# Autodesk Inventor assembly: kamerica
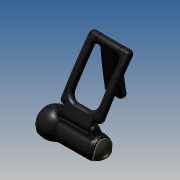
[picture p0: Inventor's stored thumbnail of the model, 180x180]
Saved by Autodesk Inventor 2012 (Build 160160000, 160)
## iProperties
Created: 2011-11-30
Part Number: kamerica
Document SubType Name: Assembly
Designer: slazh bliskovic
Author: slazh bliskovic
## Documents named in this file (12)
- C:\Users\BOZIDAR\Documents\Inventor\quickcam pro 9000\kamerica.iam
- C:\Users\BOZIDAR\Documents\Inventor\quickcam pro 9000\kamerica.ipt
- C:\Users\BOZIDAR\Documents\Inventor\quickcam pro 9000\gornji shiny dio.ipt
- C:\Users\BOZIDAR\Documents\Inventor\quickcam pro 9000\objektiv.ipt
- C:\Users\BOZIDAR\Documents\Inventor\quickcam pro 9000\unutrasnja plastika.ipt
- C:\Users\BOZIDAR\Documents\Inventor\quickcam pro 9000\staklence.ipt
- C:\Users\BOZIDAR\Documents\Inventor\quickcam pro 9000\svjetlasce.ipt
- C:\Users\BOZIDAR\Documents\Inventor\quickcam pro 9000\staklo.ipt
- C:\Users\BOZIDAR\Documents\Inventor\Content Center Files\R2012\en-US\IFI 513(1)\IFI 513 - M2x0,4 x 5(1) I.ipt
- C:\Users\BOZIDAR\Documents\Inventor\quickcam pro 9000\drska.iam
- C:\Users\BOZIDAR\Documents\Inventor\quickcam pro 9000\majk_Shrinkwrap.ipt
- C:\Users\BOZIDAR\Documents\Inventor\quickcam pro 9000\mrezica.ipt
## Components (11 placed, 11 different names)
1. kamerica:1 — Mate:1, Mate:2, Mate:3, Mate:5, Mate:6
2. gornji shiny dio:1 — Angle:1, Flush:2, Mate:6
3. objektiv:1
4. unutrasnja plastika:1
5. staklence:1 — Flush:1
6. svjetlasce:1
7. staklo:1 — Flush:1
8. Cross Recessed Flat Countersunk Head Machine Screw - Type I - Metric M2x0,4 x 5:1 — Mate:1
9. drska:1 [sub-assembly] — Mate:2, Mate:3
10. majk_Shrinkwrap:1 — Mate:5, Flush:2, Mate:7, Flush:3
11. mrezica:1 — Mate:7, Flush:3
## Relationships (11: Mate 7, Flush 3, Angle 1)
- Flush:1 (0.5 mm): staklence:1 ↔ staklo:1
- Mate:1: kamerica:1 ↔ Cross Recessed Flat Countersunk Head Machine Screw - Type I - Metric M2x0,4 x 5:1
- Mate:2: kamerica:1 ↔ drska:1
- Mate:3: kamerica:1 ↔ drska:1
- Mate:4
- Angle:1 (12.5 deg): gornji shiny dio:1
- Mate:5: kamerica:1 ↔ majk_Shrinkwrap:1
- Flush:2: gornji shiny dio:1 ↔ majk_Shrinkwrap:1
- Mate:6: kamerica:1 ↔ gornji shiny dio:1
- Mate:7: majk_Shrinkwrap:1 ↔ mrezica:1
- Flush:3 (0.5 mm): majk_Shrinkwrap:1 ↔ mrezica:1
